# Autodesk Inventor assembly: CL4-400-GB
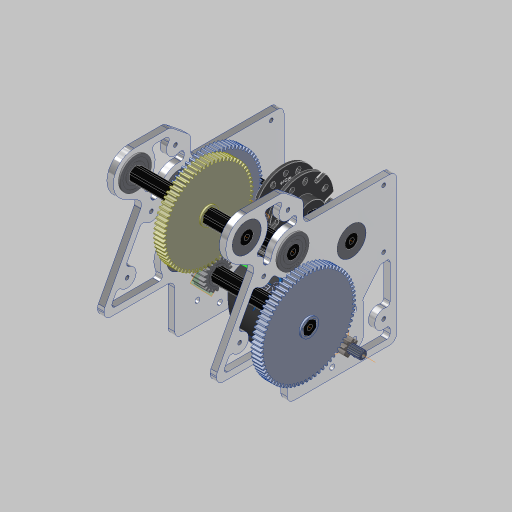
[picture p0: Inventor's stored thumbnail of the model, 512x512]
Saved by Autodesk Inventor 2023.5 (Build 275446000, 446)
## iProperties
Created: 2025-02-08
Part Number: CL4-400-GB
Document SubType Name: Assembly
Designer: slick
Mass: 1317.22 g
Surface Area: 2022.83 cm^2
Volume: 570.049 cm^3
Density: 2.31072 g/cm^3
Author: slick
## Documents named in this file (14)
- C:\Users\slick\OneDrive\Desktop\2025-ReefScape---CAD\Climber\CL4\CL4-400-GB.iam
- C:\Users\slick\OneDrive\Desktop\2025-ReefScape---CAD\Climber\CL4\CL4-016.ipt
- C:\Users\slick\OneDrive\Desktop\2025-ReefScape---CAD\COMMON PARTS\BEARINGS\0_500_ID_x_1_125_OD_x_0_313_WD_Flanged_Bearing_217-2731.ipt
- C:\Users\slick\OneDrive\Desktop\2025-ReefScape---CAD\COMMON PARTS\MOTORS\Kracken with Cover and Boards.iam
- C:\Users\slick\OneDrive\Desktop\2025-ReefScape---CAD\COMMON PARTS\GEARS\WCP-1006\WCP-1006.ipt
- C:\Users\slick\OneDrive\Desktop\2025-ReefScape---CAD\COMMON PARTS\GEARS\20dp .5 hex\72t_Aluminum_Spur_Gear_20_DP_1_2_Hex_Bore_217-3576.ipt
- C:\Users\slick\OneDrive\Desktop\2025-ReefScape---CAD\COMMON PARTS\GEARS\20dp .5 hex\20t_Aluminum_Spur_Gear_20_DP_1_2_Hex_Bore_217-2702.ipt
- C:\Users\slick\OneDrive\Desktop\2025-ReefScape---CAD\COMMON PARTS\GEARS\20dp .5 hex\68t_Aluminum_Spur_Gear_20_DP_1_2_Hex_Bore_217-5477.ipt
- C:\Users\slick\OneDrive\Desktop\2025-ReefScape---CAD\STEP files\WCP-0577\WCP-0577.ipt
- C:\Users\slick\OneDrive\Desktop\2025-ReefScape---CAD\Climber\CL4\CL4-018.ipt
- C:\Users\slick\OneDrive\Desktop\2025-ReefScape---CAD\Climber\CL4\CL4-019.ipt
- C:\Users\slick\OneDrive\Desktop\2025-ReefScape---CAD\COMMON PARTS\BEARINGS\13_75mm_1_2_ThunderHex_ID_x_1_125_OD_x_0_313_WD_Flanged_Bearing_217-4006_MIR.ipt
- C:\Users\slick\OneDrive\Desktop\2025-ReefScape---CAD\Climber\CL4\CL4-020.ipt
- C:\Users\slick\OneDrive\Desktop\2025-ReefScape---CAD\COMMON PARTS\HUBS\WCP-1388.ipt
## Components (24 placed, 13 different names)
1. CL4-016:1 — Mate:1, Mate:2, Mate:3, Mate:4, Symmetry:1, Mate:19, Mate:20, Insert:8, Insert:14, Insert:15, Insert:17
2. CL4-016:2 — Mate:1, Mate:2, Mate:3, Symmetry:1, Insert:11, Insert:12, Insert:13, Mate:27, Insert:16, Mate:34
3. 0_500_ID_x_1_125_OD_x_0_313_WD_Flanged_Bearing_217-2731:1 — Insert:12, Mate:26, Flush:6
4. 0_500_ID_x_1_125_OD_x_0_313_WD_Flanged_Bearing_217-2731:2 — Mate:16, Insert:13, Mate:23, Flush:4
5. 0_500_ID_x_1_125_OD_x_0_313_WD_Flanged_Bearing_217-2731:3 — Mate:12, Insert:11, Mate:24, Flush:5
6. 0_500_ID_x_1_125_OD_x_0_313_WD_Flanged_Bearing_217-2731:5 — Mate:14, Insert:14, Mate:28
7. 0_500_ID_x_1_125_OD_x_0_313_WD_Flanged_Bearing_217-2731:6 — Insert:8
8. Kracken with Cover and Boards:1 [sub-assembly] — Mate:4, Mate:6, Mate:7, Mate:19
9. WCP-1006:1 — Mate:6, Mate:7
10. 72t_Aluminum_Spur_Gear_20_DP_1_2_Hex_Bore_217-3576:1 — Mate:11, Mate:20, Mate:25
11. 20t_Aluminum_Spur_Gear_20_DP_1_2_Hex_Bore_217-2702:1 — Mate:11, Flush:1
12. 72t_Aluminum_Spur_Gear_20_DP_1_2_Hex_Bore_217-3576:2 — Mate:12, Flush:1, Mate:13, Mate:22
13. 20t_Aluminum_Spur_Gear_20_DP_1_2_Hex_Bore_217-2702:2 — Mate:13, Flush:2, Mate:22
14. 68t_Aluminum_Spur_Gear_20_DP_1_2_Hex_Bore_217-5477:1 — Mate:14, Flush:2, Mate:28
15. WCP-0577:1 — Mate:16, Mate:27
16. CL4-018:1 — Mate:23, Flush:4
17. CL4-019:1 — Mate:24, Flush:5
18. 13_75mm_1_2_ThunderHex_ID_x_1_125_OD_x_0_313_WD_Flanged_Bearing_217-4006_MIR:1 — Insert:15, Mate:25
19. CL4-020:1 — Mate:26, Flush:6
20. 0_500_ID_x_1_125_OD_x_0_313_WD_Flanged_Bearing_217-2731:7 — Insert:16
21. 0_500_ID_x_1_125_OD_x_0_313_WD_Flanged_Bearing_217-2731:8 — Insert:17, Mate:29, Flush:7
22. CL4-019:2 — Mate:29, Flush:7, Mate:32, Mate:33
23. WCP-1388:1 — Mate:30, Mate:31, Mate:34
24. WCP-1388:2 — Mate:30, Mate:31, Mate:32, Mate:33
## Relationships (42: Mate 26, Insert 8, Flush 7, Symmetry 1)
- Mate:1: CL4-016:1 ↔ CL4-016:2
- Mate:2: CL4-016:1 ↔ CL4-016:2
- Mate:3 (104.775 mm): CL4-016:1 ↔ CL4-016:2
- Mate:4: CL4-016:1 ↔ Kracken with Cover and Boards:1
- Mate:6: Kracken with Cover and Boards:1 ↔ WCP-1006:1
- Mate:7: Kracken with Cover and Boards:1 ↔ WCP-1006:1
- Mate:11: 72t_Aluminum_Spur_Gear_20_DP_1_2_Hex_Bore_217-3576:1 ↔ 20t_Aluminum_Spur_Gear_20_DP_1_2_Hex_Bore_217-2702:1
- Mate:12: 0_500_ID_x_1_125_OD_x_0_313_WD_Flanged_Bearing_217-2731:3 ↔ 72t_Aluminum_Spur_Gear_20_DP_1_2_Hex_Bore_217-3576:2
- Flush:1: 20t_Aluminum_Spur_Gear_20_DP_1_2_Hex_Bore_217-2702:1 ↔ 72t_Aluminum_Spur_Gear_20_DP_1_2_Hex_Bore_217-3576:2
- Mate:13: 72t_Aluminum_Spur_Gear_20_DP_1_2_Hex_Bore_217-3576:2 ↔ 20t_Aluminum_Spur_Gear_20_DP_1_2_Hex_Bore_217-2702:2
- Mate:14: 0_500_ID_x_1_125_OD_x_0_313_WD_Flanged_Bearing_217-2731:5 ↔ 68t_Aluminum_Spur_Gear_20_DP_1_2_Hex_Bore_217-5477:1
- Flush:2: 20t_Aluminum_Spur_Gear_20_DP_1_2_Hex_Bore_217-2702:2 ↔ 68t_Aluminum_Spur_Gear_20_DP_1_2_Hex_Bore_217-5477:1
- Mate:16: 0_500_ID_x_1_125_OD_x_0_313_WD_Flanged_Bearing_217-2731:2 ↔ WCP-0577:1
- Symmetry:1: CL4-016:1 ↔ CL4-016:2
- Flush:3
- Mate:19: CL4-016:1 ↔ Kracken with Cover and Boards:1
- Mate:20 (3.175 mm): CL4-016:1 ↔ 72t_Aluminum_Spur_Gear_20_DP_1_2_Hex_Bore_217-3576:1
- Insert:8: CL4-016:1 ↔ 0_500_ID_x_1_125_OD_x_0_313_WD_Flanged_Bearing_217-2731:6
- Insert:11: CL4-016:2 ↔ 0_500_ID_x_1_125_OD_x_0_313_WD_Flanged_Bearing_217-2731:3
- Insert:12: CL4-016:2 ↔ 0_500_ID_x_1_125_OD_x_0_313_WD_Flanged_Bearing_217-2731:1
- Insert:13: CL4-016:2 ↔ 0_500_ID_x_1_125_OD_x_0_313_WD_Flanged_Bearing_217-2731:2
- Insert:14: CL4-016:1 ↔ 0_500_ID_x_1_125_OD_x_0_313_WD_Flanged_Bearing_217-2731:5
- Mate:22 (25.4 mm): 72t_Aluminum_Spur_Gear_20_DP_1_2_Hex_Bore_217-3576:2 ↔ 20t_Aluminum_Spur_Gear_20_DP_1_2_Hex_Bore_217-2702:2
- Mate:23: 0_500_ID_x_1_125_OD_x_0_313_WD_Flanged_Bearing_217-2731:2 ↔ CL4-018:1
- Flush:4: 0_500_ID_x_1_125_OD_x_0_313_WD_Flanged_Bearing_217-2731:2 ↔ CL4-018:1
- Mate:24: 0_500_ID_x_1_125_OD_x_0_313_WD_Flanged_Bearing_217-2731:3 ↔ CL4-019:1
- Flush:5: 0_500_ID_x_1_125_OD_x_0_313_WD_Flanged_Bearing_217-2731:3 ↔ CL4-019:1
- Insert:15: CL4-016:1 ↔ 13_75mm_1_2_ThunderHex_ID_x_1_125_OD_x_0_313_WD_Flanged_Bearing_217-4006_MIR:1
- Mate:25: 72t_Aluminum_Spur_Gear_20_DP_1_2_Hex_Bore_217-3576:1 ↔ 13_75mm_1_2_ThunderHex_ID_x_1_125_OD_x_0_313_WD_Flanged_Bearing_217-4006_MIR:1
- Mate:26: 0_500_ID_x_1_125_OD_x_0_313_WD_Flanged_Bearing_217-2731:1 ↔ CL4-020:1
- Flush:6: 0_500_ID_x_1_125_OD_x_0_313_WD_Flanged_Bearing_217-2731:1 ↔ CL4-020:1
- Mate:27 (44.45 mm): CL4-016:2 ↔ WCP-0577:1
- Mate:28 (28.575 mm): 0_500_ID_x_1_125_OD_x_0_313_WD_Flanged_Bearing_217-2731:5 ↔ 68t_Aluminum_Spur_Gear_20_DP_1_2_Hex_Bore_217-5477:1
- Insert:16: CL4-016:2 ↔ 0_500_ID_x_1_125_OD_x_0_313_WD_Flanged_Bearing_217-2731:7
- Insert:17: CL4-016:1 ↔ 0_500_ID_x_1_125_OD_x_0_313_WD_Flanged_Bearing_217-2731:8
- Mate:29: 0_500_ID_x_1_125_OD_x_0_313_WD_Flanged_Bearing_217-2731:8 ↔ CL4-019:2
- Flush:7: 0_500_ID_x_1_125_OD_x_0_313_WD_Flanged_Bearing_217-2731:8 ↔ CL4-019:2
- Mate:30: WCP-1388:1 ↔ WCP-1388:2
- Mate:31 (12.7 mm): WCP-1388:1 ↔ WCP-1388:2
- Mate:32: CL4-019:2 ↔ WCP-1388:2
- Mate:33: CL4-019:2 ↔ WCP-1388:2
- Mate:34 (42.8625 mm): CL4-016:2 ↔ WCP-1388:1
